# Autodesk Inventor assembly: 00_003_COXA_R1
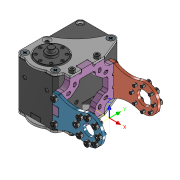
[picture p0: Inventor's stored thumbnail of the model, 180x180]
Saved by Autodesk Inventor 2021.2 (Build 252289000, 289)
## iProperties
Created: 2018-04-27
Part Number: 00_003_COXA_R1
Material: 一般
Document SubType Name: Assembly
Designer: cmflab
Mass: 88.3973 g
Surface Area: 206.931 cm^2
Volume: 50.433 cm^3
Density: 1.75277 g/cm^3
Author: cmflab
## Documents named in this file (10)
- C:\Workspace\HaptHexa\Hardware\Inventor\00_003_COXA_R1.iam
- C:\Workspace\HaptHexa\Hardware\Inventor\16_009_COXA_FRAME_4_R1.ipt
- C:\Workspace\HaptHexa\Hardware\Inventor\16_008_COXA_FRAME_3_R1.ipt
- C:\Workspace\HaptHexa\Hardware\Inventor\16_006_COXA_FRAME_1_R1.ipt
- C:\Workspace\HaptHexa\Hardware\Inventor\16_007_COXA_FRAME_2_R1.ipt
- C:\Workspace\HaptHexa\Hardware\Inventor\16_046_COXA_FRAME_5_R1.ipt
- C:\Workspace\HaptHexa\Hardware\Inventor\20_001_DYNAMIXEL_X430_R1.ipt
- C:\Workspace\HaptHexa\Hardware\Inventor\10_049_FLAT_HEAD_SCREW_M2_5X15_R1.ipt
- C:\Workspace\HaptHexa\Hardware\Inventor\10_050_CAP_BOLT_M2X6_R1.ipt
- C:\Workspace\HaptHexa\Hardware\Inventor\10_048_CAP_SCREW_M2X4_R1.ipt
## Components (36 placed, 9 different names)
1. 16_009_COXA_FRAME_4_R1:1 — メイト:3, メイト:4, メイト:5, メイト:7, メイト:8, メイト:9, メイト:15, メイト:16, メイト:17, フラッシュ:1, フラッシュ:2, Insert:1, Mate:21
2. 16_008_COXA_FRAME_3_R1:2 — メイト:4, メイト:5, メイト:3, メイト:13, Insert:8, Insert:9, Insert:12
3. 16_006_COXA_FRAME_1_R1:1 — メイト:7, メイト:8, メイト:9, Mate:22, Mate:23, Mate:24, Insert:3, Insert:4, Insert:5, Insert:6, Insert:7
4. 16_007_COXA_FRAME_2_R1:1 — メイト:15, メイト:16, メイト:17
5. 16_046_COXA_FRAME_5_R1:1 — Insert:1, Mate:21, Insert:10, Insert:11, Insert:13
6. 20_001_DYNAMIXEL_X430_R1:1 — Mate:22, Mate:23, Mate:24
7. 10_049_FLAT_HEAD_SCREW_M2_5X15_R1:1 — Insert:4
8. 10_049_FLAT_HEAD_SCREW_M2_5X15_R1:2 — Insert:3
9. 10_049_FLAT_HEAD_SCREW_M2_5X15_R1:3 — Insert:5
10. 10_049_FLAT_HEAD_SCREW_M2_5X15_R1:4
11. 10_049_FLAT_HEAD_SCREW_M2_5X15_R1:5
12. 10_049_FLAT_HEAD_SCREW_M2_5X15_R1:6
13. 10_050_CAP_BOLT_M2X6_R1:1 — Insert:6
14. 10_050_CAP_BOLT_M2X6_R1:2 — Insert:7
15. 10_050_CAP_BOLT_M2X6_R1:3 — Insert:8
16. 10_050_CAP_BOLT_M2X6_R1:4 — Insert:9
17. 10_050_CAP_BOLT_M2X6_R1:5
18. 10_050_CAP_BOLT_M2X6_R1:6
19. 10_050_CAP_BOLT_M2X6_R1:7 — Insert:10
20. 10_050_CAP_BOLT_M2X6_R1:8 — Insert:11
21. 10_048_CAP_SCREW_M2X4_R1:1 — Insert:12
22. 10_048_CAP_SCREW_M2X4_R1:2 — Insert:13
23. 10_048_CAP_SCREW_M2X4_R1:3
24. 10_048_CAP_SCREW_M2X4_R1:4
25. 10_048_CAP_SCREW_M2X4_R1:5
26. 10_048_CAP_SCREW_M2X4_R1:6
27. 10_048_CAP_SCREW_M2X4_R1:7
28. 10_048_CAP_SCREW_M2X4_R1:8
29. 10_048_CAP_SCREW_M2X4_R1:9
30. 10_048_CAP_SCREW_M2X4_R1:10
31. 10_048_CAP_SCREW_M2X4_R1:11
32. 10_048_CAP_SCREW_M2X4_R1:12
33. 10_048_CAP_SCREW_M2X4_R1:13
34. 10_048_CAP_SCREW_M2X4_R1:14
35. 10_048_CAP_SCREW_M2X4_R1:15
36. 10_048_CAP_SCREW_M2X4_R1:16
## Component patterns: (8 elements, first: 10_048_CAP_SCREW_M2X4_R1:1 + 10_048_CAP_SCREW_M2X4_R1:2)
## Relationships (28: Mate 14, Insert 12, Flush 2)
- メイト:3 [Mate]: 16_009_COXA_FRAME_4_R1:1 ↔ 16_008_COXA_FRAME_3_R1:2
- メイト:4 [Mate]: 16_009_COXA_FRAME_4_R1:1 ↔ 16_008_COXA_FRAME_3_R1:2
- メイト:5 [Mate]: 16_009_COXA_FRAME_4_R1:1 ↔ 16_008_COXA_FRAME_3_R1:2
- メイト:7 [Mate]: 16_009_COXA_FRAME_4_R1:1 ↔ 16_006_COXA_FRAME_1_R1:1
- メイト:8 [Mate]: 16_009_COXA_FRAME_4_R1:1 ↔ 16_006_COXA_FRAME_1_R1:1
- メイト:9 [Mate]: 16_009_COXA_FRAME_4_R1:1 ↔ 16_006_COXA_FRAME_1_R1:1
- メイト:13 [Mate]: 16_008_COXA_FRAME_3_R1:2
- メイト:15 [Mate]: 16_009_COXA_FRAME_4_R1:1 ↔ 16_007_COXA_FRAME_2_R1:1
- メイト:16 [Mate]: 16_009_COXA_FRAME_4_R1:1 ↔ 16_007_COXA_FRAME_2_R1:1
- メイト:17 [Mate]: 16_009_COXA_FRAME_4_R1:1 ↔ 16_007_COXA_FRAME_2_R1:1
- フラッシュ:1 [Flush] (6 mm): 16_009_COXA_FRAME_4_R1:1
- フラッシュ:2 [Flush]: 16_009_COXA_FRAME_4_R1:1
- Insert:1: 16_009_COXA_FRAME_4_R1:1 ↔ 16_046_COXA_FRAME_5_R1:1
- Mate:21: 16_009_COXA_FRAME_4_R1:1 ↔ 16_046_COXA_FRAME_5_R1:1
- Mate:22: 16_006_COXA_FRAME_1_R1:1 ↔ 20_001_DYNAMIXEL_X430_R1:1
- Mate:23: 16_006_COXA_FRAME_1_R1:1 ↔ 20_001_DYNAMIXEL_X430_R1:1
- Mate:24: 16_006_COXA_FRAME_1_R1:1 ↔ 20_001_DYNAMIXEL_X430_R1:1
- Insert:3: 16_006_COXA_FRAME_1_R1:1 ↔ 10_049_FLAT_HEAD_SCREW_M2_5X15_R1:2
- Insert:4: 16_006_COXA_FRAME_1_R1:1 ↔ 10_049_FLAT_HEAD_SCREW_M2_5X15_R1:1
- Insert:5: 16_006_COXA_FRAME_1_R1:1 ↔ 10_049_FLAT_HEAD_SCREW_M2_5X15_R1:3
- Insert:6: 16_006_COXA_FRAME_1_R1:1 ↔ 10_050_CAP_BOLT_M2X6_R1:1
- Insert:7: 16_006_COXA_FRAME_1_R1:1 ↔ 10_050_CAP_BOLT_M2X6_R1:2
- Insert:8: 16_008_COXA_FRAME_3_R1:2 ↔ 10_050_CAP_BOLT_M2X6_R1:3
- Insert:9: 16_008_COXA_FRAME_3_R1:2 ↔ 10_050_CAP_BOLT_M2X6_R1:4
- Insert:10: 16_046_COXA_FRAME_5_R1:1 ↔ 10_050_CAP_BOLT_M2X6_R1:7
- Insert:11: 16_046_COXA_FRAME_5_R1:1 ↔ 10_050_CAP_BOLT_M2X6_R1:8
- Insert:12: 16_008_COXA_FRAME_3_R1:2 ↔ 10_048_CAP_SCREW_M2X4_R1:1
- Insert:13: 16_046_COXA_FRAME_5_R1:1 ↔ 10_048_CAP_SCREW_M2X4_R1:2
## Named parameters: sa_0 = 50, sa_1 = 2e-13, sa_2 = 500, sa_3 = 0
note: some values were not read from the file. Shown as the stored number, unit unknown: "sa_0", "sa_1", "sa_2", "sa_3".
